# Autodesk Inventor assembly: panelD_onFrame
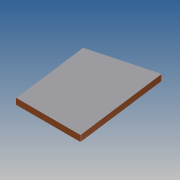
[picture p0: Inventor's stored thumbnail of the model, 180x180]
Saved by Autodesk Inventor 2014 SP1 (Build 180222100, 222)
## iProperties
Created: 2015-04-29
Part Number: panelD_onFrame
Document SubType Name: Assembly
Designer: Dave
Author: Dave
## Documents named in this file (3)
- C:\Users\Dave\Desktop\hera-cad\surface\panels\panelD_onFrame.iam
- C:\Users\Dave\Desktop\hera-cad\surface\panels\panelDframe.ipt
- C:\Users\Dave\Desktop\hera-cad\surface\panels\panelDflat.ipt
## Components (2 placed, 2 different names)
1. panelDframe:1 — Mate:1, Flush:1, Flush:2
2. panelDflat:1 — Mate:1, Flush:1, Flush:2
## Relationships (3: Flush 2, Mate 1)
- Mate:1: panelDframe:1 ↔ panelDflat:1
- Flush:1: panelDframe:1 ↔ panelDflat:1
- Flush:2: panelDframe:1 ↔ panelDflat:1
